# Autodesk Inventor assembly: Air Release 1764
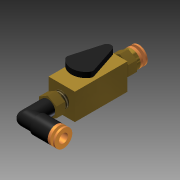
[picture p0: Inventor's stored thumbnail of the model, 180x180]
Saved by Autodesk Inventor 2011 (Build 150239000, 239)
## iProperties
Created: 2010-02-22
Part Number: Air Release 1764
Document SubType Name: Assembly
Designer: jgehrig
Author: jgehrig
## Documents named in this file (5)
- R:\CAD Archives\Pneumatics\Air Release 1764\Air Release 1764.iam
- R:\CAD Archives\Pneumatics\Air Release 1764\Air Release Base 1764.ipt
- R:\CAD Archives\Pneumatics\Air Release 1764\Knob 1764.ipt
- R:\CAD Archives\Pneumatics\Air Release 1764\Pneumatic Screw 1764\Pneumatic Screw 1764.iam
- R:\CAD Archives\Pneumatics\Air Release 1764\Pneumatics Bend Piece 1764\Pneumatic Bend Piece 1764.iam
## Components (4 placed, 4 different names)
1. Air Release Base 1764:1 — Insert:1, Insert:2, Insert:3, Angle:1
2. Knob 1764:1 — Insert:1
3. Pneumatic Screw 1764:1 [sub-assembly] — Insert:2
4. Pneumatic Bend Piece 1764:1 [sub-assembly] — Insert:3, Angle:1
## Relationships (4: Insert 3, Angle 1)
- Insert:1: Air Release Base 1764:1 ↔ Knob 1764:1
- Insert:2 (3.81 mm): Air Release Base 1764:1 ↔ Pneumatic Screw 1764:1
- Insert:3 (3.81 mm): Air Release Base 1764:1 ↔ Pneumatic Bend Piece 1764:1
- Angle:1 (0 deg): Air Release Base 1764:1 ↔ Pneumatic Bend Piece 1764:1
